# Autodesk Inventor assembly: Custom_Delta_Assembly
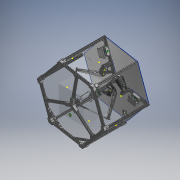
[picture p0: Inventor's stored thumbnail of the model, 180x180]
Saved by Autodesk Inventor 2019.4 (Build 234330000, 330)
## iProperties
Created: 2019-07-06
Part Number: Custom_Delta_Assembly
Document SubType Name: Assembly
Designer: Jorian Brusind
Author: Jorian Brusind
## Documents named in this file (31)
- C:\Users\Jorian Brusind\Documents\GitHub\ECE44x_Senior_Design\Design files\Delta Robot Arm\Inventor Files\Custom_Delta\Custom_Delta_Assembly.iam
- C:\Users\Jorian Brusind\Documents\GitHub\ECE44x_Senior_Design\Design files\Delta Robot Arm\Inventor Files\Custom_Delta\Stepper_Face.ipt
- C:\Users\Jorian Brusind\Documents\GitHub\ECE44x_Senior_Design\Design files\Delta Robot Arm\Inventor Files\Custom_Delta\Delta_Arm.ipt
- C:\Users\Jorian Brusind\Documents\GitHub\ECE44x_Senior_Design\Design files\Delta Robot Arm\Inventor Files\McMaster Files\5537T518_T-SLOTTED FRAMING.ipt
- C:\Users\Jorian Brusind\Documents\GitHub\ECE44x_Senior_Design\Design files\Delta Robot Arm\Inventor Files\Custom_Delta\NEMA17_Stepper_CL42H60.ipt
- C:\Users\Jorian Brusind\Documents\GitHub\ECE44x_Senior_Design\Design files\Delta Robot Arm\Inventor Files\SparkFun Files\Stepper_Collar\products\12196\step\model.ipt
- C:\Users\Jorian Brusind\Documents\GitHub\ECE44x_Senior_Design\Design files\Delta Robot Arm\Inventor Files\Custom_Delta\Workarea.ipt
- C:\Users\Jorian Brusind\Documents\GitHub\ECE44x_Senior_Design\Design files\Delta Robot Arm\Inventor Files\Custom_Delta\Frame_Skeleton.iam
- C:\Users\Jorian Brusind\Documents\GitHub\ECE44x_Senior_Design\Design files\Delta Robot Arm\Inventor Files\Custom_Delta\350mm_2020_tslot.ipt
- C:\Users\Jorian Brusind\Documents\GitHub\ECE44x_Senior_Design\Design files\Delta Robot Arm\Inventor Files\Custom_Delta\80_20_top_connector.ipt
- C:\Users\Jorian Brusind\Documents\GitHub\ECE44x_Senior_Design\Design files\Delta Robot Arm\Inventor Files\McMaster Files\98861A050_LOW-STRENGTH STEEL THREADED ROD.ipt
- C:\Users\Jorian Brusind\Documents\GitHub\ECE44x_Senior_Design\Design files\Delta Robot Arm\Inventor Files\McMaster Files\59935K140_METRIC BALL JOINT ROD END.ipt
- C:\Users\Jorian Brusind\Documents\GitHub\ECE44x_Senior_Design\Design files\Delta Robot Arm\Inventor Files\Custom_Delta\End_Effector.iam
- C:\Users\Jorian Brusind\Documents\GitHub\ECE44x_Senior_Design\Design files\Delta Robot Arm\Inventor Files\Custom_Delta\77mm_2020_tslot.ipt
- C:\Users\Jorian Brusind\Documents\GitHub\ECE44x_Senior_Design\Design files\Delta Robot Arm\Inventor Files\Custom_Delta\275mm_2020_tslot.ipt
- C:\Users\Jorian Brusind\Documents\GitHub\ECE44x_Senior_Design\Design files\Delta Robot Arm\Inventor Files\Custom_Delta\Acrylic_bottom.ipt
- C:\Users\Jorian Brusind\Documents\GitHub\ECE44x_Senior_Design\Design files\Delta Robot Arm\Inventor Files\Custom_Delta\Motor_Node.iam
- C:\Users\Jorian Brusind\Documents\GitHub\ECE44x_Senior_Design\Design files\Delta Robot Arm\Inventor Files\Metric bolt\Bolt M3 50mm.ipt
- C:\Users\Jorian Brusind\Documents\GitHub\ECE44x_Senior_Design\Design files\Delta Robot Arm\Inventor Files\Custom_Delta\120deg_Tslot_Gusset.ipt
- C:\Users\Jorian Brusind\Documents\GitHub\ECE44x_Senior_Design\Design files\Delta Robot Arm\Inventor Files\Custom_Delta\80_20_bot_connector.ipt
- C:\Users\Jorian Brusind\Documents\GitHub\ECE44x_Senior_Design\Design files\Delta Robot Arm\Inventor Files\Custom_Delta\Acrylic_bottom_camera.ipt
- C:\Users\Jorian Brusind\Documents\GitHub\ECE44x_Senior_Design\Design files\Delta Robot Arm\Inventor Files\Digikey Files\raspberry-pi-camera-module-v2-1.snapshot.3\RspCameraMia.iam
- C:\Users\Jorian Brusind\Documents\GitHub\ECE44x_Senior_Design\Design files\Delta Robot Arm\Inventor Files\Custom_Delta\Acrylic_top.ipt
- C:\Users\Jorian Brusind\Documents\GitHub\ECE44x_Senior_Design\Design files\Delta Robot Arm\Inventor Files\Custom_Delta\Limit_Switch_Bracket.ipt
- C:\Users\Jorian Brusind\Documents\GitHub\ECE44x_Senior_Design\Design files\Delta Robot Arm\Inventor Files\endstop-mechanical-limit-switch-on-pcb-1.snapshot.1\Switch.ipt
- C:\Users\Jorian Brusind\Documents\GitHub\ECE44x_Senior_Design\Design files\Delta Robot Arm\Inventor Files\Custom_Delta\Upper_Rod_Spacer.ipt
- C:\Users\Jorian Brusind\Documents\GitHub\ECE44x_Senior_Design\Design files\Delta Robot Arm\Inventor Files\Custom_Delta\Lower_Rod_Spacer.ipt
- C:\Users\Jorian Brusind\Documents\GitHub\ECE44x_Senior_Design\Design files\Delta Robot Arm\Inventor Files\Custom_Delta\Rod_constraint.ipt
- C:\Users\Jorian Brusind\Documents\GitHub\ECE44x_Senior_Design\Design files\Delta Robot Arm\Inventor Files\Custom_Delta\End_Joint_Reciever.ipt
- C:\Users\Jorian Brusind\Documents\GitHub\ECE44x_Senior_Design\Design files\Delta Robot Arm\Inventor Files\Custom_Delta\End_Joint_Rod.ipt
- C:\Users\Jorian Brusind\Documents\GitHub\ECE44x_Senior_Design\Design files\Delta Robot Arm\Inventor Files\Metric bolt\Bolt M3 20mm.ipt
## Components (78 placed, 30 different names)
1. Stepper_Face:1 — Mate:210, Mate:211, Mate:212, Mate:216, Mate:493, Flush:5, Flush:9, Mate:506, Mate:555
2. Delta_Arm:1 — Mate:214, Mate:215, Mate:254, Mate:641, Mate:643, Mate:645, Mate:654
3. Stepper_Face:2 — Mate:222, Mate:227, Mate:230, Mate:231, Mate:491, Flush:10, Mate:505, Mate:553
4. Delta_Arm:2 — Mate:220, Mate:221, Mate:253, Mate:513, Mate:514, Mate:515, Mate:516
5. Stepper_Face:3 — Mate:217, Mate:218, Mate:226, Mate:228, Mate:495, Flush:8, Mate:507, Mate:557
6. Delta_Arm:3 — Mate:224, Mate:225, Mate:229, Mate:509, Mate:510, Mate:511, Mate:512
7. NEMA17_Stepper_CL42H60:1 — Mate:219, Mate:227, Mate:230, Mate:231
8. NEMA17_Stepper_CL42H60:2 — Mate:210, Mate:211, Mate:212, Mate:213
9. NEMA17_Stepper_CL42H60:3 — Mate:217, Mate:218, Mate:223, Mate:228
10. model:4 — Mate:223, Mate:224, Mate:225, Mate:226, Mate:229
11. model:5 — Mate:213, Mate:214, Mate:215, Mate:216, Mate:254
12. model:6 — Mate:219, Mate:220, Mate:221, Mate:222, Mate:253
13. 5537T518_T-SLOTTED FRAMING:4 — Mate:500, Mate:501, Flush:11
14. 5537T518_T-SLOTTED FRAMING:5 — Mate:496, Mate:497, Flush:13
15. 5537T518_T-SLOTTED FRAMING:6 — Mate:498, Mate:499, Flush:12
16. Workarea:1 — Flush:17, Mate:558
17. Frame_Skeleton:1 [sub-assembly] — Flush:1, Mate:490, Flush:2, Mate:492, Flush:3, Flush:4, Flush:6, Flush:7, Mate:494, Mate:496, Mate:498, Mate:500, Mate:508, Flush:11, Flush:12, Flush:13, Flush:17, Mate:559, Mate:560, Flush:18, Mate:561, Flush:19, Mate:562, Mate:563, Flush:20, Mate:564, Mate:569, Mate:570, Mate:574, Mate:576, Mate:578, Mate:581, Mate:582, Mate:593, Flush:24, Mate:594, Mate:596, Mate:598, Mate:599, Mate:600, Flush:27, Mate:603, Mate:605, Mate:606, Mate:608
18. 350mm_2020_tslot:1 — Flush:6, Flush:7, Mate:494, Mate:495, Flush:8, Mate:497, Mate:556, Flush:16, Mate:577, Flush:21, Mate:618, Flush:33, Mate:627
19. 350mm_2020_tslot:2 — Flush:1, Mate:490, Flush:2, Mate:491, Mate:501, Mate:502, Mate:503, Mate:504, Flush:10, Mate:552, Flush:14, Mate:579, Flush:22, Mate:625, Flush:34
20. 350mm_2020_tslot:3 — Mate:492, Flush:3, Flush:4, Mate:493, Flush:5, Flush:9, Mate:499, Mate:554, Flush:15, Mate:580, Flush:23, Flush:32
21. 80_20_top_connector:1 — Mate:502, Mate:503, Mate:504, Mate:505, Mate:506, Mate:507, Mate:545, Mate:558
22. 98861A050_LOW-STRENGTH STEEL THREADED ROD:1 — Mate:531, Mate:532, Mate:543, Mate:544
23. 98861A050_LOW-STRENGTH STEEL THREADED ROD:2 — Mate:529, Mate:530, Mate:541, Mate:542
24. 98861A050_LOW-STRENGTH STEEL THREADED ROD:3 — Mate:537, Mate:538, Mate:639, Mate:652, Mate:653
25. 98861A050_LOW-STRENGTH STEEL THREADED ROD:4 — Mate:521, Mate:522, Mate:539, Mate:540
26. 98861A050_LOW-STRENGTH STEEL THREADED ROD:5 — Mate:535, Mate:536, Mate:630, Mate:631, Mate:633, Mate:636, Mate:638, Mate:646, Mate:651
27. 98861A050_LOW-STRENGTH STEEL THREADED ROD:6 — Mate:523, Mate:524, Mate:533, Mate:534
28. 59935K140_METRIC BALL JOINT ROD END:2 — Mate:535, Mate:536, Mate:551, Mate:634
29. 59935K140_METRIC BALL JOINT ROD END:3 — Mate:511, Mate:512, Mate:521, Mate:522, Mate:591
30. 59935K140_METRIC BALL JOINT ROD END:4 — Mate:509, Mate:510, Mate:523, Mate:524, Mate:592
31. 59935K140_METRIC BALL JOINT ROD END:5 — Mate:537, Mate:538, Mate:550
32. 59935K140_METRIC BALL JOINT ROD END:6 — Mate:515, Mate:516, Mate:531, Mate:532, Mate:589
33. 59935K140_METRIC BALL JOINT ROD END:7 — Mate:513, Mate:514, Mate:529, Mate:530, Mate:590
34. 59935K140_METRIC BALL JOINT ROD END:8 — Mate:543, Mate:544, Mate:546
35. 59935K140_METRIC BALL JOINT ROD END:9 — Mate:541, Mate:542, Mate:547
36. 59935K140_METRIC BALL JOINT ROD END:11 — Mate:533, Mate:534, Mate:549
37. 59935K140_METRIC BALL JOINT ROD END:12 — Mate:539, Mate:540, Mate:548
38. End_Effector:1 [sub-assembly] — Mate:545, Mate:546, Mate:547, Mate:548, Mate:549, Mate:550, Mate:551
39. 77mm_2020_tslot:1 — Mate:552, Flush:14, Mate:553
40. 77mm_2020_tslot:2 — Mate:554, Flush:15, Mate:555
41. 77mm_2020_tslot:3 — Mate:556, Flush:16, Mate:557
42. 275mm_2020_tslot:1 — Mate:559, Mate:560, Flush:18, Mate:575, Mate:604, Flush:30, Mate:607, Flush:31, Mate:610, Mate:611
43. 275mm_2020_tslot:2 — Mate:561, Flush:19, Mate:562, Mate:595, Flush:25, Mate:597, Flush:26
44. 275mm_2020_tslot:3 — Mate:563, Flush:20, Mate:564, Mate:568, Mate:601, Mate:602, Flush:28, Flush:29, Mate:609, Mate:613
45. Acrylic_bottom:1 — Mate:568, Mate:569, Mate:570, Mate:612, Mate:614
46. Acrylic_bottom:3 — Mate:574, Mate:575, Mate:576
47. Motor_Node:1 [sub-assembly] — Mate:577, Mate:578, Flush:21
48. Motor_Node:2 [sub-assembly] — Mate:579, Mate:581, Flush:22
49. Motor_Node:3 [sub-assembly] — Mate:580, Mate:582, Flush:23
50. Bolt M3 50mm:1 — Mate:641, Mate:642, Mate:643, Mate:644
51. Bolt M3 50mm:2 — Mate:589, Mate:590
52. Bolt M3 50mm:3 — Mate:591, Mate:592
53. 120deg_Tslot_Gusset:1 — Mate:593, Flush:24, Mate:594
54. 120deg_Tslot_Gusset:2 — Mate:599, Mate:600, Flush:27
55. 5537T518_T-SLOTTED FRAMING:7 — Mate:597, Mate:598, Flush:26
56. 5537T518_T-SLOTTED FRAMING:8 — Mate:595, Mate:596, Flush:25
57. 5537T518_T-SLOTTED FRAMING:9 — Mate:607, Mate:608, Flush:31
58. 5537T518_T-SLOTTED FRAMING:10 — Mate:604, Mate:605, Flush:30
59. 5537T518_T-SLOTTED FRAMING:11 — Mate:602, Mate:603, Flush:29
60. 5537T518_T-SLOTTED FRAMING:12 — Mate:601, Mate:606, Flush:28
61. 80_20_bot_connector:1 — Mate:609, Mate:610, Mate:611
62. Acrylic_bottom_camera:1 — Mate:612, Mate:613, Mate:614, Mate:615, Mate:616, Mate:617
63. RspCameraMia:1 [sub-assembly] — Mate:615, Mate:616, Mate:617
64. Acrylic_top:1 — Mate:618, Flush:32, Flush:33, Mate:619, Mate:620, Mate:621, Mate:626, Mate:629
65. Limit_Switch_Bracket:1 — Mate:619, Mate:620, Mate:621, Mate:622, Mate:623, Mate:624
66. Switch:1 — Mate:622, Mate:623, Mate:624
67. Acrylic_top:2 — Mate:627, Mate:628, Mate:629
68. Acrylic_top:3 — Mate:625, Mate:626, Flush:34, Mate:628
69. Upper_Rod_Spacer:1 — Mate:630, Mate:632, Mate:635
70. Upper_Rod_Spacer:2 — Mate:631, Mate:632, Mate:640
71. Lower_Rod_Spacer:1 — Mate:633, Mate:634, Mate:635
72. Lower_Rod_Spacer:2 — Mate:636, Mate:648
73. Rod_constraint:1 — Mate:638, Mate:639, Mate:640
74. End_Joint_Reciever:1 — Mate:642, Mate:654, Mate:656
75. End_Joint_Rod:1 — Mate:646, Mate:648, Mate:650, Mate:651, Mate:655, Mate:657, Mate:658
76. End_Joint_Reciever:2 — Mate:644, Mate:645, Mate:650, Mate:655
77. End_Joint_Rod:2 — Mate:652, Mate:653, Mate:656
78. Bolt M3 20mm:1 — Mate:657, Mate:658
## Relationships (204: Mate 170, Flush 34)
- Mate:210: Stepper_Face:1 ↔ NEMA17_Stepper_CL42H60:2
- Mate:211: Stepper_Face:1 ↔ NEMA17_Stepper_CL42H60:2
- Mate:212: Stepper_Face:1 ↔ NEMA17_Stepper_CL42H60:2
- Mate:213: NEMA17_Stepper_CL42H60:2 ↔ model:5
- Mate:214: Delta_Arm:1 ↔ model:5
- Mate:215: Delta_Arm:1 ↔ model:5
- Mate:216: Stepper_Face:1 ↔ model:5
- Mate:217: Stepper_Face:3 ↔ NEMA17_Stepper_CL42H60:3
- Mate:218: Stepper_Face:3 ↔ NEMA17_Stepper_CL42H60:3
- Mate:219: NEMA17_Stepper_CL42H60:1 ↔ model:6
- Mate:220: Delta_Arm:2 ↔ model:6
- Mate:221: Delta_Arm:2 ↔ model:6
- Mate:222: Stepper_Face:2 ↔ model:6
- Mate:223: NEMA17_Stepper_CL42H60:3 ↔ model:4
- Mate:224: Delta_Arm:3 ↔ model:4
- Mate:225: Delta_Arm:3 ↔ model:4
- Mate:226: Stepper_Face:3 ↔ model:4
- Mate:227: Stepper_Face:2 ↔ NEMA17_Stepper_CL42H60:1
- Mate:228: Stepper_Face:3 ↔ NEMA17_Stepper_CL42H60:3
- Mate:229: Delta_Arm:3 ↔ model:4
- Mate:230: Stepper_Face:2 ↔ NEMA17_Stepper_CL42H60:1
- Mate:231: Stepper_Face:2 ↔ NEMA17_Stepper_CL42H60:1
- Mate:253: Delta_Arm:2 ↔ model:6
- Mate:254: Delta_Arm:1 ↔ model:5
- Flush:1: Frame_Skeleton:1 ↔ 350mm_2020_tslot:2
- Mate:490: Frame_Skeleton:1 ↔ 350mm_2020_tslot:2
- Flush:2: Frame_Skeleton:1 ↔ 350mm_2020_tslot:2
- Mate:491: Stepper_Face:2 ↔ 350mm_2020_tslot:2
- Mate:492: Frame_Skeleton:1 ↔ 350mm_2020_tslot:3
- Flush:3: Frame_Skeleton:1 ↔ 350mm_2020_tslot:3
- Flush:4: Frame_Skeleton:1 ↔ 350mm_2020_tslot:3
- Mate:493: Stepper_Face:1 ↔ 350mm_2020_tslot:3
- Flush:5: Stepper_Face:1 ↔ 350mm_2020_tslot:3
- Flush:6: Frame_Skeleton:1 ↔ 350mm_2020_tslot:1
- Flush:7: Frame_Skeleton:1 ↔ 350mm_2020_tslot:1
- Mate:494: Frame_Skeleton:1 ↔ 350mm_2020_tslot:1
- Mate:495: Stepper_Face:3 ↔ 350mm_2020_tslot:1
- Flush:8: Stepper_Face:3 ↔ 350mm_2020_tslot:1
- Flush:9: Stepper_Face:1 ↔ 350mm_2020_tslot:3
- Mate:496: 5537T518_T-SLOTTED FRAMING:5 ↔ Frame_Skeleton:1
- Mate:497: 5537T518_T-SLOTTED FRAMING:5 ↔ 350mm_2020_tslot:1
- Mate:498: 5537T518_T-SLOTTED FRAMING:6 ↔ Frame_Skeleton:1
- Mate:499: 5537T518_T-SLOTTED FRAMING:6 ↔ 350mm_2020_tslot:3
- Mate:500: 5537T518_T-SLOTTED FRAMING:4 ↔ Frame_Skeleton:1
- Mate:501: 5537T518_T-SLOTTED FRAMING:4 ↔ 350mm_2020_tslot:2
- Mate:502: 350mm_2020_tslot:2 ↔ 80_20_top_connector:1
- Mate:503 (0.5 mm): 350mm_2020_tslot:2 ↔ 80_20_top_connector:1
- Mate:504 (0.5 mm): 350mm_2020_tslot:2 ↔ 80_20_top_connector:1
- Flush:10: Stepper_Face:2 ↔ 350mm_2020_tslot:2
- Mate:505 (120 mm): Stepper_Face:2 ↔ 80_20_top_connector:1
- Mate:506 (120 mm): Stepper_Face:1 ↔ 80_20_top_connector:1
- Mate:507 (120 mm): Stepper_Face:3 ↔ 80_20_top_connector:1
- Mate:508: Frame_Skeleton:1
- Flush:11: 5537T518_T-SLOTTED FRAMING:4 ↔ Frame_Skeleton:1
- Flush:12: 5537T518_T-SLOTTED FRAMING:6 ↔ Frame_Skeleton:1
- Flush:13: 5537T518_T-SLOTTED FRAMING:5 ↔ Frame_Skeleton:1
- Mate:509: Delta_Arm:3 ↔ 59935K140_METRIC BALL JOINT ROD END:4
- Mate:510 (10 mm): Delta_Arm:3 ↔ 59935K140_METRIC BALL JOINT ROD END:4
- Mate:511: Delta_Arm:3 ↔ 59935K140_METRIC BALL JOINT ROD END:3
- Mate:512 (10 mm): Delta_Arm:3 ↔ 59935K140_METRIC BALL JOINT ROD END:3
- Mate:513: Delta_Arm:2 ↔ 59935K140_METRIC BALL JOINT ROD END:7
- Mate:514 (10 mm): Delta_Arm:2 ↔ 59935K140_METRIC BALL JOINT ROD END:7
- Mate:515: Delta_Arm:2 ↔ 59935K140_METRIC BALL JOINT ROD END:6
- Mate:516 (10 mm): Delta_Arm:2 ↔ 59935K140_METRIC BALL JOINT ROD END:6
- Mate:521: 98861A050_LOW-STRENGTH STEEL THREADED ROD:4 ↔ 59935K140_METRIC BALL JOINT ROD END:3
- Mate:522: 98861A050_LOW-STRENGTH STEEL THREADED ROD:4 ↔ 59935K140_METRIC BALL JOINT ROD END:3
- Mate:523: 98861A050_LOW-STRENGTH STEEL THREADED ROD:6 ↔ 59935K140_METRIC BALL JOINT ROD END:4
- Mate:524: 98861A050_LOW-STRENGTH STEEL THREADED ROD:6 ↔ 59935K140_METRIC BALL JOINT ROD END:4
- Mate:529: 98861A050_LOW-STRENGTH STEEL THREADED ROD:2 ↔ 59935K140_METRIC BALL JOINT ROD END:7
- Mate:530: 98861A050_LOW-STRENGTH STEEL THREADED ROD:2 ↔ 59935K140_METRIC BALL JOINT ROD END:7
- Mate:531: 98861A050_LOW-STRENGTH STEEL THREADED ROD:1 ↔ 59935K140_METRIC BALL JOINT ROD END:6
- Mate:532: 98861A050_LOW-STRENGTH STEEL THREADED ROD:1 ↔ 59935K140_METRIC BALL JOINT ROD END:6
- Mate:533: 98861A050_LOW-STRENGTH STEEL THREADED ROD:6 ↔ 59935K140_METRIC BALL JOINT ROD END:11
- Mate:534 (-10 mm): 98861A050_LOW-STRENGTH STEEL THREADED ROD:6 ↔ 59935K140_METRIC BALL JOINT ROD END:11
- Mate:535: 98861A050_LOW-STRENGTH STEEL THREADED ROD:5 ↔ 59935K140_METRIC BALL JOINT ROD END:2
- Mate:536 (-10 mm): 98861A050_LOW-STRENGTH STEEL THREADED ROD:5 ↔ 59935K140_METRIC BALL JOINT ROD END:2
- Mate:537: 98861A050_LOW-STRENGTH STEEL THREADED ROD:3 ↔ 59935K140_METRIC BALL JOINT ROD END:5
- Mate:538 (-10 mm): 98861A050_LOW-STRENGTH STEEL THREADED ROD:3 ↔ 59935K140_METRIC BALL JOINT ROD END:5
- Mate:539: 98861A050_LOW-STRENGTH STEEL THREADED ROD:4 ↔ 59935K140_METRIC BALL JOINT ROD END:12
- Mate:540 (-10 mm): 98861A050_LOW-STRENGTH STEEL THREADED ROD:4 ↔ 59935K140_METRIC BALL JOINT ROD END:12
- Mate:541: 98861A050_LOW-STRENGTH STEEL THREADED ROD:2 ↔ 59935K140_METRIC BALL JOINT ROD END:9
- Mate:542 (-10 mm): 98861A050_LOW-STRENGTH STEEL THREADED ROD:2 ↔ 59935K140_METRIC BALL JOINT ROD END:9
- Mate:543: 98861A050_LOW-STRENGTH STEEL THREADED ROD:1 ↔ 59935K140_METRIC BALL JOINT ROD END:8
- Mate:544 (-10 mm): 98861A050_LOW-STRENGTH STEEL THREADED ROD:1 ↔ 59935K140_METRIC BALL JOINT ROD END:8
- Mate:545: 80_20_top_connector:1 ↔ End_Effector:1
- Mate:546: 59935K140_METRIC BALL JOINT ROD END:8 ↔ End_Effector:1
- Mate:547: 59935K140_METRIC BALL JOINT ROD END:9 ↔ End_Effector:1
- Mate:548: 59935K140_METRIC BALL JOINT ROD END:12 ↔ End_Effector:1
- Mate:549: 59935K140_METRIC BALL JOINT ROD END:11 ↔ End_Effector:1
- Mate:550: 59935K140_METRIC BALL JOINT ROD END:5 ↔ End_Effector:1
- Mate:551: 59935K140_METRIC BALL JOINT ROD END:2 ↔ End_Effector:1
- Mate:552: 350mm_2020_tslot:2 ↔ 77mm_2020_tslot:1
- Flush:14: 350mm_2020_tslot:2 ↔ 77mm_2020_tslot:1
- Mate:553: Stepper_Face:2 ↔ 77mm_2020_tslot:1
- Mate:554: 350mm_2020_tslot:3 ↔ 77mm_2020_tslot:2
- Flush:15: 350mm_2020_tslot:3 ↔ 77mm_2020_tslot:2
- Mate:555: Stepper_Face:1 ↔ 77mm_2020_tslot:2
- Mate:556: 350mm_2020_tslot:1 ↔ 77mm_2020_tslot:3
- Flush:16: 350mm_2020_tslot:1 ↔ 77mm_2020_tslot:3
- Mate:557: Stepper_Face:3 ↔ 77mm_2020_tslot:3
- Flush:17: Workarea:1 ↔ Frame_Skeleton:1
- Mate:558: Workarea:1 ↔ 80_20_top_connector:1
- Mate:559: Frame_Skeleton:1 ↔ 275mm_2020_tslot:1
- Mate:560 (140.5 mm): Frame_Skeleton:1 ↔ 275mm_2020_tslot:1
- Flush:18: Frame_Skeleton:1 ↔ 275mm_2020_tslot:1
- Mate:561: Frame_Skeleton:1 ↔ 275mm_2020_tslot:2
- Flush:19: Frame_Skeleton:1 ↔ 275mm_2020_tslot:2
- Mate:562 (140.5 mm): Frame_Skeleton:1 ↔ 275mm_2020_tslot:2
- Mate:563: Frame_Skeleton:1 ↔ 275mm_2020_tslot:3
- Flush:20: Frame_Skeleton:1 ↔ 275mm_2020_tslot:3
- Mate:564 (140.5 mm): Frame_Skeleton:1 ↔ 275mm_2020_tslot:3
- Mate:568: 275mm_2020_tslot:3 ↔ Acrylic_bottom:1
- Mate:569: Frame_Skeleton:1 ↔ Acrylic_bottom:1
- Mate:570: Frame_Skeleton:1 ↔ Acrylic_bottom:1
- Mate:574: Frame_Skeleton:1 ↔ Acrylic_bottom:3
- Mate:575: 275mm_2020_tslot:1 ↔ Acrylic_bottom:3
- Mate:576: Frame_Skeleton:1 ↔ Acrylic_bottom:3
- Mate:577: 350mm_2020_tslot:1 ↔ Motor_Node:1
- Mate:578 (60 mm): Frame_Skeleton:1 ↔ Motor_Node:1
- Flush:21 (-20 mm): 350mm_2020_tslot:1 ↔ Motor_Node:1
- Mate:579: 350mm_2020_tslot:2 ↔ Motor_Node:2
- Mate:580: 350mm_2020_tslot:3 ↔ Motor_Node:3
- Mate:581 (60 mm): Frame_Skeleton:1 ↔ Motor_Node:2
- Flush:22 (-20 mm): 350mm_2020_tslot:2 ↔ Motor_Node:2
- Mate:582 (60 mm): Frame_Skeleton:1 ↔ Motor_Node:3
- Flush:23 (-20 mm): 350mm_2020_tslot:3 ↔ Motor_Node:3
- Mate:589: 59935K140_METRIC BALL JOINT ROD END:6 ↔ Bolt M3 50mm:2
- Mate:590 (5 mm): 59935K140_METRIC BALL JOINT ROD END:7 ↔ Bolt M3 50mm:2
- Mate:591: 59935K140_METRIC BALL JOINT ROD END:3 ↔ Bolt M3 50mm:3
- Mate:592 (5 mm): 59935K140_METRIC BALL JOINT ROD END:4 ↔ Bolt M3 50mm:3
- Mate:593: Frame_Skeleton:1 ↔ 120deg_Tslot_Gusset:1
- Flush:24: Frame_Skeleton:1 ↔ 120deg_Tslot_Gusset:1
- Mate:594: Frame_Skeleton:1 ↔ 120deg_Tslot_Gusset:1
- Mate:595: 275mm_2020_tslot:2 ↔ 5537T518_T-SLOTTED FRAMING:8
- Mate:596: Frame_Skeleton:1 ↔ 5537T518_T-SLOTTED FRAMING:8
- Flush:25: 275mm_2020_tslot:2 ↔ 5537T518_T-SLOTTED FRAMING:8
- Mate:597: 275mm_2020_tslot:2 ↔ 5537T518_T-SLOTTED FRAMING:7
- Mate:598: Frame_Skeleton:1 ↔ 5537T518_T-SLOTTED FRAMING:7
- Flush:26: 275mm_2020_tslot:2 ↔ 5537T518_T-SLOTTED FRAMING:7
- Mate:599: Frame_Skeleton:1 ↔ 120deg_Tslot_Gusset:2
- Mate:600: Frame_Skeleton:1 ↔ 120deg_Tslot_Gusset:2
- Flush:27: Frame_Skeleton:1 ↔ 120deg_Tslot_Gusset:2
- Mate:601: 275mm_2020_tslot:3 ↔ 5537T518_T-SLOTTED FRAMING:12
- Mate:602: 275mm_2020_tslot:3 ↔ 5537T518_T-SLOTTED FRAMING:11
- Mate:603: Frame_Skeleton:1 ↔ 5537T518_T-SLOTTED FRAMING:11
- Mate:604: 275mm_2020_tslot:1 ↔ 5537T518_T-SLOTTED FRAMING:10
- Mate:605: Frame_Skeleton:1 ↔ 5537T518_T-SLOTTED FRAMING:10
- Mate:606: Frame_Skeleton:1 ↔ 5537T518_T-SLOTTED FRAMING:12
- Flush:28: 275mm_2020_tslot:3 ↔ 5537T518_T-SLOTTED FRAMING:12
- Flush:29: 275mm_2020_tslot:3 ↔ 5537T518_T-SLOTTED FRAMING:11
- Flush:30: 275mm_2020_tslot:1 ↔ 5537T518_T-SLOTTED FRAMING:10
- Mate:607: 275mm_2020_tslot:1 ↔ 5537T518_T-SLOTTED FRAMING:9
- Mate:608: Frame_Skeleton:1 ↔ 5537T518_T-SLOTTED FRAMING:9
- Flush:31: 275mm_2020_tslot:1 ↔ 5537T518_T-SLOTTED FRAMING:9
- Mate:609 (5 mm): 275mm_2020_tslot:3 ↔ 80_20_bot_connector:1
- Mate:610 (5 mm): 275mm_2020_tslot:1 ↔ 80_20_bot_connector:1
- Mate:611 (1 mm): 275mm_2020_tslot:1 ↔ 80_20_bot_connector:1
- Mate:612 (4 mm): Acrylic_bottom:1 ↔ Acrylic_bottom_camera:1
- Mate:613: 275mm_2020_tslot:3 ↔ Acrylic_bottom_camera:1
- Mate:614 (2 mm): Acrylic_bottom:1 ↔ Acrylic_bottom_camera:1
- Mate:615: Acrylic_bottom_camera:1 ↔ RspCameraMia:1
- Mate:616: Acrylic_bottom_camera:1 ↔ RspCameraMia:1
- Mate:617 (10 mm): Acrylic_bottom_camera:1 ↔ RspCameraMia:1
- Mate:618: 350mm_2020_tslot:1 ↔ Acrylic_top:1
- Flush:32 (10 mm): 350mm_2020_tslot:3 ↔ Acrylic_top:1
- Flush:33 (10 mm): 350mm_2020_tslot:1 ↔ Acrylic_top:1
- Mate:619: Acrylic_top:1 ↔ Limit_Switch_Bracket:1
- Mate:620: Acrylic_top:1 ↔ Limit_Switch_Bracket:1
- Mate:621: Acrylic_top:1 ↔ Limit_Switch_Bracket:1
- Mate:622: Limit_Switch_Bracket:1 ↔ Switch:1
- Mate:623: Limit_Switch_Bracket:1 ↔ Switch:1
- Mate:624 (1 mm): Limit_Switch_Bracket:1 ↔ Switch:1
- Mate:625: 350mm_2020_tslot:2 ↔ Acrylic_top:3
- Mate:626 (1 mm): Acrylic_top:1 ↔ Acrylic_top:3
- Flush:34: 350mm_2020_tslot:2 ↔ Acrylic_top:3
- Mate:627: 350mm_2020_tslot:1 ↔ Acrylic_top:2
- Mate:628 (1 mm): Acrylic_top:2 ↔ Acrylic_top:3
- Mate:629 (1 mm): Acrylic_top:1 ↔ Acrylic_top:2
- Mate:630: 98861A050_LOW-STRENGTH STEEL THREADED ROD:5 ↔ Upper_Rod_Spacer:1
- Mate:631: 98861A050_LOW-STRENGTH STEEL THREADED ROD:5 ↔ Upper_Rod_Spacer:2
- Mate:632 (7.5 mm): Upper_Rod_Spacer:1 ↔ Upper_Rod_Spacer:2
- Mate:633: 98861A050_LOW-STRENGTH STEEL THREADED ROD:5 ↔ Lower_Rod_Spacer:1
- Mate:634: 59935K140_METRIC BALL JOINT ROD END:2 ↔ Lower_Rod_Spacer:1
- Mate:635 (7.5 mm): Upper_Rod_Spacer:1 ↔ Lower_Rod_Spacer:1
- Mate:636: 98861A050_LOW-STRENGTH STEEL THREADED ROD:5 ↔ Lower_Rod_Spacer:2
- Mate:638: 98861A050_LOW-STRENGTH STEEL THREADED ROD:5 ↔ Rod_constraint:1
- Mate:639: 98861A050_LOW-STRENGTH STEEL THREADED ROD:3 ↔ Rod_constraint:1
- Mate:640 (1 mm): Upper_Rod_Spacer:2 ↔ Rod_constraint:1
- Mate:641: Delta_Arm:1 ↔ Bolt M3 50mm:1
- Mate:642: Bolt M3 50mm:1 ↔ End_Joint_Reciever:1
- Mate:643 (22 mm): Delta_Arm:1 ↔ Bolt M3 50mm:1
- Mate:644: Bolt M3 50mm:1 ↔ End_Joint_Reciever:2
- Mate:645: Delta_Arm:1 ↔ End_Joint_Reciever:2
- Mate:646: 98861A050_LOW-STRENGTH STEEL THREADED ROD:5 ↔ End_Joint_Rod:1
- Mate:648: Lower_Rod_Spacer:2 ↔ End_Joint_Rod:1
- Mate:650: End_Joint_Rod:1 ↔ End_Joint_Reciever:2
- Mate:651: 98861A050_LOW-STRENGTH STEEL THREADED ROD:5 ↔ End_Joint_Rod:1
- Mate:652: 98861A050_LOW-STRENGTH STEEL THREADED ROD:3 ↔ End_Joint_Rod:2
- Mate:653: 98861A050_LOW-STRENGTH STEEL THREADED ROD:3 ↔ End_Joint_Rod:2
- Mate:654: Delta_Arm:1 ↔ End_Joint_Reciever:1
- Mate:655 (1 mm): End_Joint_Rod:1 ↔ End_Joint_Reciever:2
- Mate:656: End_Joint_Reciever:1 ↔ End_Joint_Rod:2
- Mate:657: End_Joint_Rod:1 ↔ Bolt M3 20mm:1
- Mate:658: End_Joint_Rod:1 ↔ Bolt M3 20mm:1
